# Autodesk Inventor assembly: Assembly1
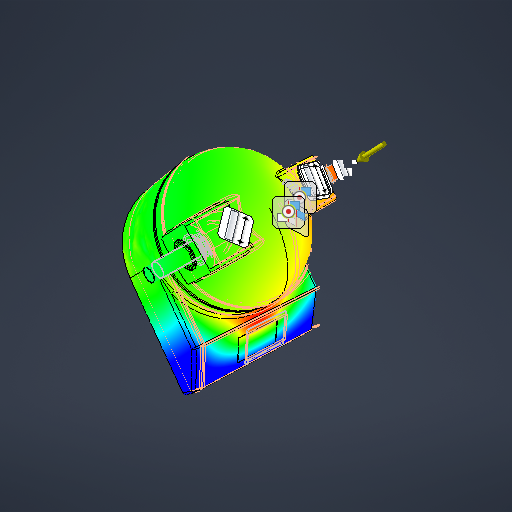
[picture p0: Inventor's stored thumbnail of the model, 512x512]
Saved by Autodesk Inventor 2025 (Build 290162000, 162)
## iProperties
Created: 2024-04-14
Part Number: Assembly1
Document SubType Name: Assembly
Designer: sicia
Mass: 1745.41 g
Surface Area: 6311.55 cm^2
Volume: 1085.28 cm^3
Density: 1.60826 g/cm^3
Author: sicia
## Documents named in this file (20)
- D:\Dokumenty\GitHub\ESP32_tracker\hardware\Assembly1.iam
- D:\Pobrane\St3020_servo\Slip Ring.ipt
- D:\Pobrane\St3020_servo\st3020 servo.iam
- D:\Dokumenty\GitHub\ESP32_tracker\hardware\Góra.ipt
- D:\Dokumenty\GitHub\ESP32_tracker\hardware\wal.ipt
- D:\Dokumenty\GitHub\ESP32_tracker\hardware\Pokrywa_góra.ipt
- D:\Pobrane\Hitec Servo Motor HS-311.ipt
- D:\Pobrane\hs-422_horn_disc_sws(1).ipt
- D:\Dokumenty\GitHub\ESP32_tracker\hardware\Assembly1\Design Accelerator\Bearing4.iam
- D:\Dokumenty\GitHub\ESP32_tracker\hardware\Assembly1\Design Accelerator\Bearing5.iam
- D:\Dokumenty\GitHub\ESP32_tracker\hardware\Assembly1\Design Accelerator\Spur Gears2.iam
- D:\Dokumenty\GitHub\ESP32_tracker\hardware\Dół.ipt
- D:\Dokumenty\GitHub\ESP32_tracker\hardware\Ekran.iam
- D:\Dokumenty\GitHub\ESP32_tracker\hardware\Assembly1\Design Accelerator\Spur Gears5.iam
- D:\Dokumenty\GitHub\ESP32_tracker\hardware\Assembly1\AIP\FEA\eo83glkww.fins
- D:\Dokumenty\GitHub\ESP32_tracker\hardware\Assembly1\AIP\FEA\eo83glkww.fsat
- D:\Dokumenty\GitHub\ESP32_tracker\hardware\Assembly1\AIP\FEA\eo83glkww.ftes
- D:\Dokumenty\GitHub\ESP32_tracker\hardware\Assembly1\AIP\FEA\eo83glkww.fwiz
- D:\Dokumenty\GitHub\ESP32_tracker\hardware\Assembly1\AIP\FEA\eo83gll28.fmsh
- D:\Dokumenty\GitHub\ESP32_tracker\hardware\Assembly1\AIP\FEA\eo83gll29.fres
## Components (13 placed, 11 different names)
1. Slip Ring:1
2. st3020 servo:1 [sub-assembly] — Rigid:7, Mate:15, Mate:16
3. Góra:1 — Rigid:8, Rotational:3, Rotational:4
4. wal:1 — Mate:8, Mate:10, Mate:11, Mate:14
5. Pokrywa_góra:1 — Rigid:4, Rigid:8, Rotational:2, Mate:17
6. Hitec Servo Motor HS-311:1 — Rigid:4, Rotational:1
7. hs-422_horn_disc_sws(1):1 — Rotational:1, Mate:12, Mate:13
8. Bearing:1 [sub-assembly] — Mate:8, Rotational:3
9. Bearing:2 [sub-assembly] — Mate:10, Mate:11, Rotational:4
10. Spur Gears:1 [sub-assembly] — Mate:12, Mate:13, Mate:14
11. Dół:1 — Rigid:5, Rigid:7, Rotational:2
12. Ekran:1 [sub-assembly] — Rigid:5
13. Spur Gears:2 [sub-assembly] — Mate:15, Mate:16, Mate:17
## Relationships (17: Mate 9, WeldJoint 4, RevoluteJoint 4)
- Mate:8: wal:1 ↔ Bearing:1
- Mate:10: wal:1 ↔ Bearing:2
- Mate:11 (-50 mm): wal:1 ↔ Bearing:2
- Rigid:4 [WeldJoint]: Pokrywa_góra:1 ↔ Hitec Servo Motor HS-311:1
- Rotational:1 [RevoluteJoint]: Hitec Servo Motor HS-311:1 ↔ hs-422_horn_disc_sws(1):1
- Mate:12: hs-422_horn_disc_sws(1):1 ↔ Spur Gears:1
- Mate:13: hs-422_horn_disc_sws(1):1 ↔ Spur Gears:1
- Mate:14: wal:1 ↔ Spur Gears:1
- Rigid:5 [WeldJoint]: Dół:1 ↔ Ekran:1
- Rigid:7 [WeldJoint]: st3020 servo:1 ↔ Dół:1
- Rigid:8 [WeldJoint]: Góra:1 ↔ Pokrywa_góra:1
- Rotational:2 [RevoluteJoint]: Pokrywa_góra:1 ↔ Dół:1
- Mate:15: st3020 servo:1 ↔ Spur Gears:2
- Mate:16: st3020 servo:1 ↔ Spur Gears:2
- Mate:17: Pokrywa_góra:1 ↔ Spur Gears:2
- Rotational:3 [RevoluteJoint]: Góra:1 ↔ Bearing:1
- Rotational:4 [RevoluteJoint]: Góra:1 ↔ Bearing:2
## Named parameters: sa_0 = -10000, sa_1 = -10000, sa_2 = 0
note: some values were not read from the file. Shown as the stored number, unit unknown: "sa_0", "sa_1", "sa_2".
